# Autodesk Inventor assembly: prueba4
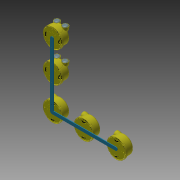
[picture p0: Inventor's stored thumbnail of the model, 180x180]
Saved by Autodesk Inventor 2015 (Build 190159000, 159)
## iProperties
Created: 2015-06-07
Part Number: prueba4
Document SubType Name: Assembly
Designer: david_000
Author: david_000
## Documents named in this file (3)
- C:\Users\david_000\Desktop\minibot-code\mechanics\prueba4.iam
- C:\Users\david_000\Desktop\minibot-code\mechanics\suelo_pruebas.ipt
- C:\Users\david_000\Desktop\minibot-code\mechanics\minibot.iam
## Components (6 placed, 2 different names)
1. suelo_pruebas:1 — Coincidencia:1, Coincidencia:2, Coincidencia:3, Coincidencia:4, Ángulo:1
2. minibot:1 [sub-assembly] — Coincidencia:1, Coincidencia:2, Nivelación:1, Nivelación:4
3. minibot:2 [sub-assembly] — Nivelación:1, Nivelación:2, Nivelación:3, Nivelación:4
4. minibot:3 [sub-assembly] — Nivelación:2, Coincidencia:3, Nivelación:3, Nivelación:5, Nivelación:6
5. minibot:4 [sub-assembly] — Coincidencia:4, Nivelación:5, Nivelación:7, Nivelación:8
6. minibot:5 [sub-assembly] — Nivelación:6, Nivelación:7, Nivelación:8, Ángulo:1
## Relationships (13: Flush 8, Mate 4, Angle 1)
- Coincidencia:1 [Mate]: suelo_pruebas:1 ↔ minibot:1
- Coincidencia:2 [Mate]: suelo_pruebas:1 ↔ minibot:1
- Nivelación:1 [Flush]: minibot:1 ↔ minibot:2
- Nivelación:2 [Flush]: minibot:2 ↔ minibot:3
- Coincidencia:3 [Mate]: suelo_pruebas:1 ↔ minibot:3
- Nivelación:3 [Flush]: minibot:2 ↔ minibot:3
- Nivelación:4 [Flush]: minibot:1 ↔ minibot:2
- Coincidencia:4 [Mate]: suelo_pruebas:1 ↔ minibot:4
- Nivelación:5 [Flush]: minibot:3 ↔ minibot:4
- Nivelación:6 [Flush]: minibot:3 ↔ minibot:5
- Nivelación:7 [Flush]: minibot:4 ↔ minibot:5
- Nivelación:8 [Flush]: minibot:4 ↔ minibot:5
- Ángulo:1 [Angle] (0 deg): suelo_pruebas:1 ↔ minibot:5
